# Autodesk Inventor assembly: head_new
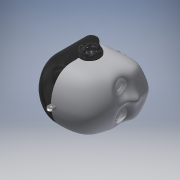
[picture p0: Inventor's stored thumbnail of the model, 180x180]
Saved by Autodesk Inventor 2019 (Build 230136000, 136)
## iProperties
Created: 2015-02-23
Part Number: head_new
Document SubType Name: Assembly
Designer: 4mahboob
Mass: 294.137 g
Surface Area: 2481.5 cm^2
Volume: 294.137 cm^3
Density: 1 g/cm^3
Sending System: SolidWorks 2014
Last Author: 4mahboob
Author: 4mahboob
## Documents named in this file (5)
- Z:\NICO_CAD\NICO-CAD\Nico_CAD_N\Nico_N\Head_N\head_new.iam
- Z:\Nico_N\NICO-CAD-master\NICO_CAD_master\head\Hinterkopf.ipt
- Z:\NICO_CAD\NICO-CAD\Nico_CAD_N\Nico_N\Head_N\iCub_Head_new.ipt
- Z:\NICO_CAD\NICO-CAD\Nico_CAD_N\Nico_N\Head_N\ear_right_cut.ipt
- Z:\NICO_CAD\NICO-CAD\Nico_CAD_N\Nico_N\Head_N\ear_right_cut_MIR.ipt
## Components (4 placed, 4 different names)
1. Hinterkopf:1 — Mate:1, Mate:2, Mate:3, Mate:4
2. iCub_Head_new:1 — Mate:1, Mate:2, Mate:3
3. ear_right_cut:1 — Mate:4
4. ear_right_cut_MIR:1
## Relationships (4: Mate 4)
- Mate:1: Hinterkopf:1 ↔ iCub_Head_new:1
- Mate:2: Hinterkopf:1 ↔ iCub_Head_new:1
- Mate:3 (-51.5 mm): Hinterkopf:1 ↔ iCub_Head_new:1
- Mate:4: Hinterkopf:1 ↔ ear_right_cut:1
